# Autodesk Inventor assembly: Outer Channel Right
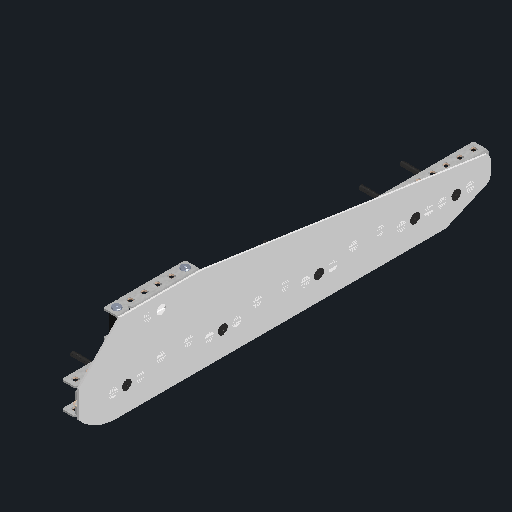
[picture p0: Inventor's stored thumbnail of the model, 512x512]
Saved by Autodesk Inventor 2025 (Build 290162000, 162)
## iProperties
Created: 2024-10-17
Part Number: Outer Channel Right
Document SubType Name: Assembly
Designer: Averey Ku
Author: averey
## Documents named in this file (22)
- D:\VEX\High Stakes\CAD\V2\Chassis\Drivebay Right\Outer Channel Right.iam
- D:\VEX\High Stakes\CAD\V2\Chassis\Drivebay Right\Bearing Flat NScrew Slotted Right.iam
- D:\VEX\High Stakes\CAD\V2\Chassis\Drivebay Right\ASScrew Hex Threaded 2.000 Right.ipt
- D:\VEX\High Stakes\CAD\V2\Chassis\Drivebay Right\Alu C 1x2x1x30 Right.ipt
- D:\VEX\High Stakes\CAD\V2\Chassis\Drivebay Right\Alu C 1x2x1x6 Right.ipt
- D:\VEX\High Stakes\CAD\ROBOPROS-CAD-Inventor\Motion\Spacers\Spacer Nylon .500 OD\NSpacer White .500 OD x .500.ipt
- D:\VEX\High Stakes\CAD\V2\Chassis\Drivebay Right\Bearing Flat NScrew Slotted Offset Right.iam
- D:\VEX\High Stakes\CAD\V2\Chassis\Drivebay Right\Skirt Right.ipt
- D:\VEX\High Stakes\CAD\ROBOPROS-CAD-Inventor\Motion\Spacers\Spacer Nylon .375 OD\NSpacer .375 OD x .875.ipt
- D:\VEX\High Stakes\CAD\V2\Chassis\Drivebay Right\Nut Keps Right.ipt
- D:\VEX\High Stakes\CAD\ROBOPROS-CAD-Inventor\Structure\Standoff\Standoff .875.ipt
- D:\VEX\High Stakes\CAD\ROBOPROS-CAD-Inventor\Structure\Hardware\Screw Steel - Star\SScrew Star Smooth 1.750.ipt
- D:\VEX\High Stakes\CAD\ROBOPROS-CAD-Inventor\Structure\Hardware\Screw Steel - Star\SScrew Star Smooth .290.ipt
- D:\VEX\High Stakes\CAD\V2\Chassis\Drivebay Right\Bearing Flat Low Profile Right.ipt
- D:\VEX\High Stakes\CAD\ROBOPROS-CAD-Inventor\Structure\Hardware\Screw Shoulder Robosource\SScrew Shoulder Smooth 2.000 x .04.ipt
- D:\VEX\High Stakes\CAD\ROBOPROS-CAD-Inventor\Structure\Hardware\Nut Nylon\Nut Nylon - White.ipt
- C:\Users\avere\VEX\High Stakes\CAD\ROBOPROS-CAD-Inventor\Motion\Spacers\Spacer Nylon .500 OD.ipt
- C:\Users\avere\VEX\High Stakes\CAD\ROBOPROS-CAD-Inventor\Motion\Spacers\Spacer Nylon .375 OD.ipt
- C:\Users\avere\VEX\High Stakes\CAD\ROBOPROS-CAD-Inventor\Structure\Standoff.ipt
- C:\Users\avere\VEX\High Stakes\CAD\ROBOPROS-CAD-Inventor\Structure\Hardware\Screw Steel - Star.ipt
- C:\Users\avere\VEX\High Stakes\CAD\ROBOPROS-CAD-Inventor\Structure\Hardware\Screw Shoulder Robosource.ipt
- C:\Users\avere\VEX\High Stakes\CAD\ROBOPROS-CAD-Inventor\Structure\Hardware\Nut Nylon.ipt
## Components (30 placed, 15 different names)
1. Alu C 1x2x1x30 Right:1 — Mate:1, Mate:4, Insert:3, Mate:5, Insert:4, Mate:6, Insert:5, Insert:6, Insert:7, Insert:9, Insert:10, Insert:16, Insert:15, Insert:18, Insert:22, Mate:9, Insert:23
2. Alu C 1x2x1x6 Right:1 — Insert:8, Insert:13, Insert:17, Insert:19, Insert:24, Insert:22, Mate:9
3. NSpacer White .500 OD x .500:1 — Insert:9, Insert:8
4. NSpacer White .500 OD x .500:2 — Insert:10, Mate:8
5. Bearing Flat NScrew Slotted Offset Right:1 [sub-assembly] — Insert:22, Mate:9
6. Skirt Right:1 — Insert:12
7. NSpacer .375 OD x .875:1 — Insert:13, Mate:8
8. Nut Keps Right:1 — Insert:16
9. Nut Keps Right:2 — Insert:15
10. Standoff .875:1 — Insert:17
11. SScrew Star Smooth 1.750:1 — Insert:18
12. SScrew Star Smooth .290:2 — Insert:19
13. Standoff .875:2 — Insert:22
14. Bearing Flat Low Profile Right:1 — Mate:9, Insert:23, Insert:25, Insert:26
15. SScrew Shoulder Smooth 2.000 x .04:1 — Insert:24
16. Nut Nylon - White:1 — Insert:25
17. Nut Nylon - White:2 — Insert:26
18. Bearing Flat NScrew Slotted Right:1 [sub-assembly] — Mate:4, Insert:3
19. Bearing Flat NScrew Slotted Right:4 [sub-assembly]
20. Bearing Flat NScrew Slotted Right:2 [sub-assembly] — Mate:5, Insert:4
21. Bearing Flat NScrew Slotted Right:5 [sub-assembly]
22. Bearing Flat NScrew Slotted Right:6 [sub-assembly]
23. Bearing Flat NScrew Slotted Right:3 [sub-assembly] — Mate:6, Insert:5
24. Bearing Flat NScrew Slotted Right:7 [sub-assembly]
25. Bearing Flat NScrew Slotted Right:8 [sub-assembly]
26. ASScrew Hex Threaded 2.000 Right:1 — Insert:6, Insert:12
27. ASScrew Hex Threaded 2.000 Right:3
28. ASScrew Hex Threaded 2.000 Right:2 — Insert:7
29. ASScrew Hex Threaded 2.000 Right:4
30. ASScrew Hex Threaded 2.000 Right:5
## Component patterns: (2 elements, first: Bearing Flat NScrew Slotted Right:1), (3 elements, first: Bearing Flat NScrew Slotted Right:2), (3 elements, first: Bearing Flat NScrew Slotted Right:3), (2 elements, first: ASScrew Hex Threaded 2.000 Right:1), (3 elements, first: ASScrew Hex Threaded 2.000 Right:2)
## Relationships (28: Insert 21, Mate 7)
- Mate:1: Alu C 1x2x1x30 Right:1
- Mate:4: Alu C 1x2x1x30 Right:1 ↔ Bearing Flat NScrew Slotted Right:1
- Insert:3: Alu C 1x2x1x30 Right:1 ↔ Bearing Flat NScrew Slotted Right:1
- Mate:5: Alu C 1x2x1x30 Right:1 ↔ Bearing Flat NScrew Slotted Right:2
- Insert:4: Alu C 1x2x1x30 Right:1 ↔ Bearing Flat NScrew Slotted Right:2
- Mate:6: Alu C 1x2x1x30 Right:1 ↔ Bearing Flat NScrew Slotted Right:3
- Insert:5: Alu C 1x2x1x30 Right:1 ↔ Bearing Flat NScrew Slotted Right:3
- Insert:6 (-1.5875 mm): Alu C 1x2x1x30 Right:1 ↔ ASScrew Hex Threaded 2.000 Right:1
- Insert:7 (-1.5875 mm): Alu C 1x2x1x30 Right:1 ↔ ASScrew Hex Threaded 2.000 Right:2
- Insert:9: Alu C 1x2x1x30 Right:1 ↔ NSpacer White .500 OD x .500:1
- Insert:8: Alu C 1x2x1x6 Right:1 ↔ NSpacer White .500 OD x .500:1
- Insert:10: Alu C 1x2x1x30 Right:1 ↔ NSpacer White .500 OD x .500:2
- Insert:12: Skirt Right:1 ↔ ASScrew Hex Threaded 2.000 Right:1
- Insert:13: Alu C 1x2x1x6 Right:1 ↔ NSpacer .375 OD x .875:1
- Insert:16: Alu C 1x2x1x30 Right:1 ↔ Nut Keps Right:1
- Insert:15: Alu C 1x2x1x30 Right:1 ↔ Nut Keps Right:2
- Insert:17: Alu C 1x2x1x6 Right:1 ↔ Standoff .875:1
- Insert:18: Alu C 1x2x1x30 Right:1 ↔ SScrew Star Smooth 1.750:1
- Insert:19: Alu C 1x2x1x6 Right:1 ↔ SScrew Star Smooth .290:2
- Insert:22: Alu C 1x2x1x30 Right:1 ↔ Standoff .875:2
- Mate:9: Alu C 1x2x1x30 Right:1 ↔ Bearing Flat Low Profile Right:1
- Insert:23: Alu C 1x2x1x30 Right:1 ↔ Bearing Flat Low Profile Right:1
- Insert:24: Alu C 1x2x1x6 Right:1 ↔ SScrew Shoulder Smooth 2.000 x .04:1
- Insert:25 (1.27 mm): Bearing Flat Low Profile Right:1 ↔ Nut Nylon - White:1
- Insert:26 (1.27 mm): Bearing Flat Low Profile Right:1 ↔ Nut Nylon - White:2
- Mate:8: NSpacer White .500 OD x .500:2 ↔ NSpacer .375 OD x .875:1
- Insert:22: Alu C 1x2x1x6 Right:1 ↔ Bearing Flat NScrew Slotted Offset Right:1
- Mate:9: Alu C 1x2x1x6 Right:1 ↔ Bearing Flat NScrew Slotted Offset Right:1
